# Autodesk Inventor assembly: MAIN
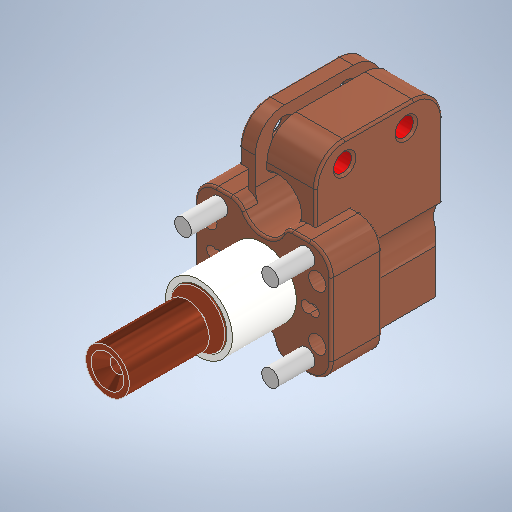
[picture p0: Inventor's stored thumbnail of the model, 512x512]
Saved by Autodesk Inventor 2025.3 (Build 293356030, 356C)
## iProperties
Created: 2025-08-19
Part Number: MAIN
Document SubType Name: Assembly
Designer: wangg
Author: wangg
## iProperties of the stored document MemberDocs/xLywjz3rtIcuwmtglBtgtivlzFh
Created: 2025-08-19
Part Number: MAIN
Document SubType Name: Assembly
Designer: wangg
Author: wangg
## Documents named in this file (19)
- C:\Users\plebbb\Desktop\Crazy_Dragon_LC\MAIN.iam
- C:\Users\plebbb\Desktop\Crazy_Dragon_LC\Purchased Parts\NF-Crazy Volcano heat block\NF-Crazy Volcano heat block\NF-Crazy Volcano heat block.ipt
- C:\Users\plebbb\Desktop\Crazy_Dragon_LC\Purchased Parts\Creality Spider Pro\Creality Spider Pro\Creality Spider Pro.ipt
- C:\Users\plebbb\Desktop\Crazy_Dragon_LC\Heatsink_HOTEND_WC_CHANNEL.ipt
- C:\Users\plebbb\Desktop\Crazy_Dragon_LC\Purchased Parts\Ceramic_Spacer.ipt
- C:\Users\plebbb\Desktop\Crazy_Dragon_LC\Purchased Parts\HGX Lite Extruder\HGX Lite Extruder\6mm Bearing (1).ipt
- C:\Users\plebbb\Desktop\Crazy_Dragon_LC\Purchased Parts\HGX Lite Extruder\HGX Lite Extruder\PTFE Connector.ipt
- C:\Users\plebbb\Desktop\Crazy_Dragon_LC\Purchased Parts\HGX Lite Extruder\HGX Lite Extruder\Reduction Gear.ipt
- C:\Users\plebbb\Desktop\Crazy_Dragon_LC\Purchased Parts\HGX Lite Extruder\HGX Lite Extruder\Filament Gear.ipt
- C:\Users\plebbb\Desktop\Crazy_Dragon_LC\Purchased Parts\HGX Lite Extruder\HGX Lite Extruder\Filament Gear001.ipt
- C:\Users\plebbb\Desktop\Crazy_Dragon_LC\Purchased Parts\HGX Lite Extruder\HGX Lite Extruder\rod 16mm001.ipt
- C:\Users\plebbb\Desktop\Crazy_Dragon_LC\Purchased Parts\HGX Lite Extruder\HGX Lite Extruder\Tensioner Screw023.iam
- C:\Users\plebbb\Desktop\Crazy_Dragon_LC\Purchased Parts\HGX Lite Extruder\HGX Lite Extruder\6mm Bearing.ipt
- C:\Users\plebbb\Desktop\Crazy_Dragon_LC\Purchased Parts\HGX Lite Extruder\HGX Lite Extruder\rod 16mm.ipt
- C:\Users\plebbb\Desktop\Crazy_Dragon_LC\Purchased Parts\HGX Lite Extruder\HGX Lite Extruder\rod 24mm.ipt
- C:\Users\plebbb\Desktop\Crazy_Dragon_LC\Purchased Parts\MGN9.ipt
- C:\Users\plebbb\Desktop\Crazy_Dragon_LC\Purchased Parts\HGX Lite Extruder\HGX Lite Extruder\Motor.ipt
- C:\Users\plebbb\Desktop\Crazy_Dragon_LC\Templates\1.75mm_Filament.ipt
- C:\Users\plebbb\Desktop\Crazy_Dragon_LC\Purchased Parts\MGN9H.ipt
## Components (7 placed, 4 different names)
1. NF-Crazy Volcano heat block:1 — Mate:1, Mate:2, Mate:3, Mate:4, Mate:5, Mate:6, Mate:7, Mate:8, Mate:9, Mate:10
2. Creality Spider Pro:1 — Mate:1, Mate:2
3. Heatsink_HOTEND_WC_CHANNEL:1
4. Ceramic_Spacer:1 — Mate:4, Mate:8
5. Ceramic_Spacer:2 — Mate:3, Mate:7
6. Ceramic_Spacer:3 — Mate:5, Mate:10
7. Ceramic_Spacer:4 — Mate:6, Mate:9
## Relationships (10: Mate 10)
- Mate:1: NF-Crazy Volcano heat block:1 ↔ Creality Spider Pro:1
- Mate:2: NF-Crazy Volcano heat block:1 ↔ Creality Spider Pro:1
- Mate:3: NF-Crazy Volcano heat block:1 ↔ Ceramic_Spacer:2
- Mate:4: NF-Crazy Volcano heat block:1 ↔ Ceramic_Spacer:1
- Mate:5: NF-Crazy Volcano heat block:1 ↔ Ceramic_Spacer:3
- Mate:6: NF-Crazy Volcano heat block:1 ↔ Ceramic_Spacer:4
- Mate:7: NF-Crazy Volcano heat block:1 ↔ Ceramic_Spacer:2
- Mate:8: NF-Crazy Volcano heat block:1 ↔ Ceramic_Spacer:1
- Mate:9: NF-Crazy Volcano heat block:1 ↔ Ceramic_Spacer:4
- Mate:10: NF-Crazy Volcano heat block:1 ↔ Ceramic_Spacer:3
